# Autodesk Inventor assembly: Y_rail_Assembly_Rev3
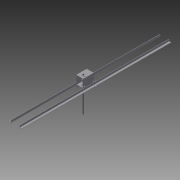
[picture p0: Inventor's stored thumbnail of the model, 180x180]
Saved by Autodesk Inventor 2015 (Build 190159000, 159)
## iProperties
Created: 2017-01-11
Part Number: Y_rail_Assembly_Rev3
Document SubType Name: Assembly
Designer: Guy
Mass: 1796.89 g
Surface Area: 4829.55 cm^2
Volume: 1200.62 cm^3
Density: 1.49664 g/cm^3
Author: Guy
## Documents named in this file (3)
- C:\Users\Guy\Documents\Fourth Year\Capstone\git\Capstone-Project\doc\CAD\LowLevel_Rev3\Y_rail_Assembly_Rev3.iam
- C:\Users\Guy\Documents\Fourth Year\Capstone\git\Capstone-Project\doc\CAD\LowLevel_Rev3\Y_Rail-SquareBar-Rev3.ipt
- C:\Users\Guy\Documents\Fourth Year\Capstone\git\Capstone-Project\doc\CAD\EndEffectorBase2\Assembly1.iam
## Components (3 placed, 2 different names)
1. Y_Rail-SquareBar-Rev3:1 — Mate:97, Mate:99, Mate:102, Angle:1, Mate:103
2. Y_Rail-SquareBar-Rev3:2 — Mate:97, Mate:99, Mate:102, Tangent:1, Tangent:2
3. Assembly1:1 [sub-assembly] — Tangent:1, Tangent:2, Mate:103
## Relationships (7: Mate 4, Tangent 2, Angle 1)
- Mate:97: Y_Rail-SquareBar-Rev3:1 ↔ Y_Rail-SquareBar-Rev3:2
- Mate:99 (97 mm): Y_Rail-SquareBar-Rev3:1 ↔ Y_Rail-SquareBar-Rev3:2
- Mate:102: Y_Rail-SquareBar-Rev3:1 ↔ Y_Rail-SquareBar-Rev3:2
- Tangent:1: Y_Rail-SquareBar-Rev3:2 ↔ Assembly1:1
- Tangent:2: Y_Rail-SquareBar-Rev3:2 ↔ Assembly1:1
- Angle:1 (0 deg): Y_Rail-SquareBar-Rev3:1
- Mate:103: Y_Rail-SquareBar-Rev3:1 ↔ Assembly1:1
